# Autodesk Inventor assembly: Geniva
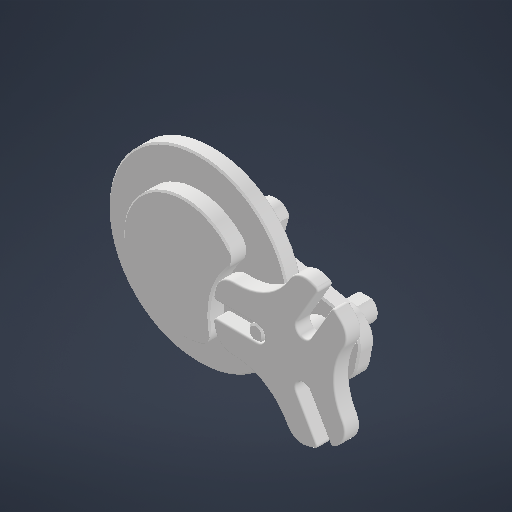
[picture p0: Inventor's stored thumbnail of the model, 512x512]
Saved by Autodesk Inventor 2026.3 (Build 303398000, 398)
## iProperties
Created: 2026-04-30
Part Number: Geniva
Document SubType Name: Assembly
Designer: frede
Author: frede
## Documents named in this file (4)
- E:\Git\AppliedAutomationProject\feeder\trayFeeder\Geniva.iam
- E:\Git\AppliedAutomationProject\feeder\trayFeeder\genivaBottom.ipt
- E:\Git\AppliedAutomationProject\feeder\trayFeeder\geniva1.ipt
- E:\Git\AppliedAutomationProject\feeder\trayFeeder\geniva2.ipt
## Components (3 placed, 3 different names)
1. genivaBottom:1 — Mate:2, Mate:3, Mate:4, Mate:5
2. geniva1:1 — Mate:2, Mate:3, Mate:6
3. geniva2:1 — Mate:4, Mate:5, Mate:6
## Relationships (5: Mate 5)
- Mate:2: genivaBottom:1 ↔ geniva1:1
- Mate:3: genivaBottom:1 ↔ geniva1:1
- Mate:4: genivaBottom:1 ↔ geniva2:1
- Mate:5: genivaBottom:1 ↔ geniva2:1
- Mate:6 (2.55 mm): geniva1:1 ↔ geniva2:1
